# Autodesk Inventor assembly: Facade16
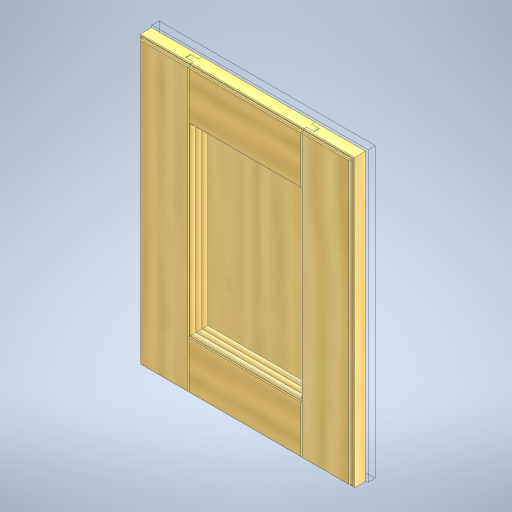
[picture p0: Inventor's stored thumbnail of the model, 512x512]
Saved by Autodesk Inventor 2024 (Build 280153000, 153)
## iProperties
RuleStatus: InUse
Created: 2019-10-02
Part Number: Facade16
Document SubType Name: Assembly
Designer: RokasM
Author: RokasM
## Documents named in this file (7)
- C:\W4INV 2024 Design\iBOX LIBRARY\Facades\Solid Wood Facade 16\Facade16.iam
- C:\W4INV 2024 Design\iBOX LIBRARY\Facades\Solid Wood Facade 16\box.ipt
- C:\W4INV 2024 Design\iBOX LIBRARY\Facades\Solid Wood Facade 16\profile_left.ipt
- C:\W4INV 2024 Design\iBOX LIBRARY\Facades\Solid Wood Facade 16\profile_right.ipt
- C:\W4INV 2024 Design\iBOX LIBRARY\Facades\Solid Wood Facade 16\profile_top.ipt
- C:\W4INV 2024 Design\iBOX LIBRARY\Facades\Solid Wood Facade 16\panel.ipt
- C:\W4INV 2024 Design\iBOX LIBRARY\Facades\Solid Wood Facade 16\Facade16.ipt
## Components (7 placed, 6 different names)
1. @Facade16
2. box:1
3. profile_left:1 — Mate:1
4. profile_right:1 — Mate:2, Flush:1
5. profile_top:1
6. panel:1
7. profile_top:2 — Mate:1, Mate:2, Flush:1
## Relationships (3: Mate 2, Flush 1)
- Mate:1: profile_left:1 ↔ profile_top:2
- Mate:2: profile_right:1 ↔ profile_top:2
- Flush:1: profile_right:1 ↔ profile_top:2
## Named parameters: offset_top = 0 mm, offset_right = 0 mm, offset_bottom = 0 mm, offset_left = 0 mm, offset_facade = 2 mm, tolerance_top = 1.5 mm, tolerance_right = 1.5 mm, tolerance_bottom = 1.5 mm, tolerance_left = 1.5 mm
